# Autodesk Inventor assembly: Model1Assembly
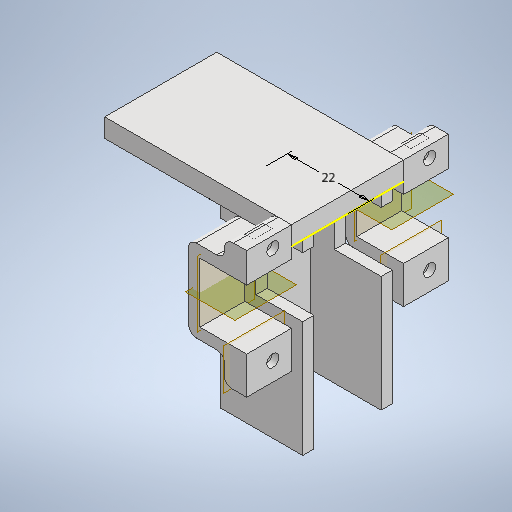
[picture p0: Inventor's stored thumbnail of the model, 512x512]
Saved by Autodesk Inventor 2025.1 (Build 291241020, 241B)
## iProperties
Created: 2025-04-14
Part Number: Model1Assembly
Document SubType Name: Assembly
Designer: omiye
Author: omiye
## Documents named in this file (4)
- C:\Projects\Arduino\sumobotV2\models\Model1Assembly.iam
- C:\Projects\Arduino\sumobotV2\models\nanoMount.ipt
- C:\Projects\Arduino\sumobotV2\models\motorMount.ipt
- C:\Projects\Arduino\sumobotV2\models\batteryMount.ipt
## Components (4 placed, 3 different names)
1. nanoMount:1 — Mate:4, Mate:5, Mate:6, Mate:10, Mate:11, Mate:12
2. motorMount:1 — Mate:11, Mate:12
3. motorMount:2 — Mate:4, Mate:10
4. batteryMount:1 — Mate:5, Mate:6
## Relationships (6: Mate 6)
- Mate:4: nanoMount:1 ↔ motorMount:2
- Mate:5: nanoMount:1 ↔ batteryMount:1
- Mate:6: nanoMount:1 ↔ batteryMount:1
- Mate:10: nanoMount:1 ↔ motorMount:2
- Mate:11: nanoMount:1 ↔ motorMount:1
- Mate:12: nanoMount:1 ↔ motorMount:1
